# Autodesk Inventor assembly: floorfitment
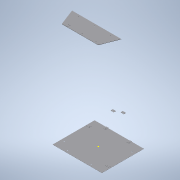
[picture p0: Inventor's stored thumbnail of the model, 180x180]
Saved by Autodesk Inventor 2021 (Build 250183000, 183)
## iProperties
Created: 2020-11-06
Part Number: floorfitment
Document SubType Name: Assembly
Designer: mackeycj
Author: mackeycj
Quantity: 1
## Documents named in this file (4)
- C:\Users\mackeycj\Downloads\floorplan2-20201106T152714Z-001\floorplan2\floorfitment.iam
- C:\Users\mackeycj\Desktop\seatfloorfit.ipt
- C:\Users\mackeycj\Desktop\mountingtabsquareshort.ipt
- C:\Users\mackeycj\Downloads\floorplan2-20201106T152714Z-001\floorplan2\angledfloorfit.ipt
## Components (10 placed, 3 different names)
1. seatfloorfit:1 — Mate:1, Angle:1, Mate:3, Mate:4, Angle:2, Mate:5, Angle:3, Mate:6, Angle:4, Mate:8
2. mountingtabsquareshort:1 — Angle:1, Mate:4
3. mountingtabsquareshort:2 — Mate:3, Angle:2
4. mountingtabsquareshort:3 — Mate:6, Angle:4
5. mountingtabsquareshort:4 — Mate:5, Angle:3
6. mountingtabsquareshort:5
7. mountingtabsquareshort:6
8. mountingtabsquareshort:7 — Mate:9
9. mountingtabsquareshort:8 — Mate:10, Angle:5
10. angledfloorfit:1 — Mate:7, Flush:1, Mate:9, Mate:10, Angle:5
## Relationships (15: Mate 9, Angle 5, Flush 1)
- Mate:1: seatfloorfit:1
- Angle:1 (0 deg): seatfloorfit:1 ↔ mountingtabsquareshort:1
- Mate:3: seatfloorfit:1 ↔ mountingtabsquareshort:2
- Mate:4: seatfloorfit:1 ↔ mountingtabsquareshort:1
- Angle:2 (0 deg): seatfloorfit:1 ↔ mountingtabsquareshort:2
- Mate:5: seatfloorfit:1 ↔ mountingtabsquareshort:4
- Angle:3 (0 deg): seatfloorfit:1 ↔ mountingtabsquareshort:4
- Mate:6: seatfloorfit:1 ↔ mountingtabsquareshort:3
- Angle:4 (0 deg): seatfloorfit:1 ↔ mountingtabsquareshort:3
- Mate:7 (1016 mm): angledfloorfit:1
- Mate:8: seatfloorfit:1
- Flush:1: angledfloorfit:1
- Mate:9: mountingtabsquareshort:7 ↔ angledfloorfit:1
- Mate:10: mountingtabsquareshort:8 ↔ angledfloorfit:1
- Angle:5 (0 deg): mountingtabsquareshort:8 ↔ angledfloorfit:1
